# Autodesk Inventor assembly: Assembly
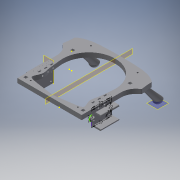
[picture p0: Inventor's stored thumbnail of the model, 180x180]
Saved by Autodesk Inventor 2019 (Build 230136000, 136)
## iProperties
Created: 2019-04-08
Part Number: Assembly
Material: Ogólny
Document SubType Name: Assembly
Designer: terg
Author: terg
## Documents named in this file (4)
- D:\Projekt\Projekt---platforma-mobilna\Chassis\Assembly.iam
- D:\Projekt\Projekt---platforma-mobilna\Chassis\base.ipt
- D:\Projekt\Projekt---platforma-mobilna\Chassis\motor_grip_L.ipt
- D:\Projekt\Projekt---platforma-mobilna\Chassis\motor_grip_R.ipt
## Components (3 placed, 3 different names)
1. base:1 — Płaskie:1, Płaskie:2
2. motor_grip_L:1 — Płaskie:1
3. motor_grip_R:1 — Płaskie:2
## Relationships (2: PlanarJoint 2)
- Płaskie:1 [PlanarJoint]: base:1 ↔ motor_grip_L:1
- Płaskie:2 [PlanarJoint]: base:1 ↔ motor_grip_R:1
